# Autodesk Inventor assembly: ToASI-5
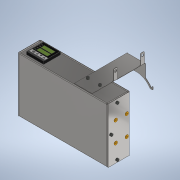
[picture p0: Inventor's stored thumbnail of the model, 180x180]
Saved by Autodesk Inventor 2020.3 (Build 243373000, 373)
## iProperties
Created: 2020-08-01
Part Number: ToASI-5
Document SubType Name: Assembly
Designer: Bruno
Author: Bruno
## Documents named in this file (4)
- C:\Users\Bruno\Desktop\Github\CAD\Inventor\For ASI\ToASI-5.iam
- C:\Users\Bruno\Desktop\Github\CAD\Inventor\For ASI\ToASI-4.iam
- C:\Users\Bruno\Desktop\Github\CAD\Inventor\Heater-Box\Glass vase _ flow meter fixer\Glass fixer plate.ipt
- C:\Users\Bruno\Desktop\Github\CAD\Inventor\Heater-Box\Glass vase _ flow meter fixer\DIN912 M4x0.7x10-8.8 socket head screw.ipt
## Components (4 placed, 3 different names)
1. ToASI-4:1 [sub-assembly] — Cylindrical:1
2. Glass fixer plate:1 — Cylindrical:1, Cylindrical:2, Cylindrical:3
3. DIN912 M4x0.7x10-8.8 socket head screw:1 — Cylindrical:3
4. DIN912 M4x0.7x10-8.8 socket head screw:2 — Cylindrical:2
## Relationships (3: CylindricalJoint 3)
- Cylindrical:1: ToASI-4:1 ↔ Glass fixer plate:1
- Cylindrical:2: Glass fixer plate:1 ↔ DIN912 M4x0.7x10-8.8 socket head screw:2
- Cylindrical:3: Glass fixer plate:1 ↔ DIN912 M4x0.7x10-8.8 socket head screw:1
